# Autodesk Inventor assembly: diagonalstretcher_MIR
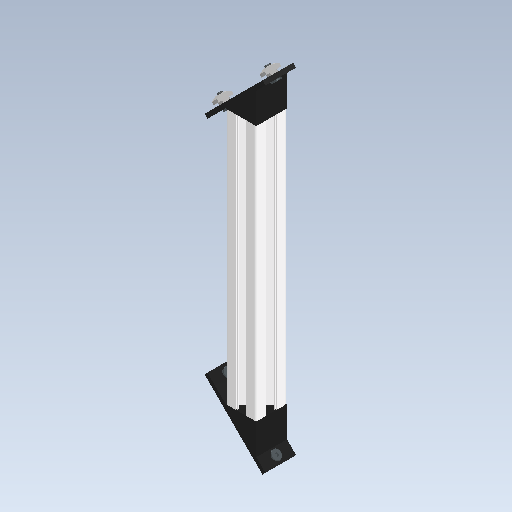
[picture p0: Inventor's stored thumbnail of the model, 512x512]
Saved by Autodesk Inventor 2020.2 (Build 242310000, 310)
## iProperties
Created: 2020-07-25
Part Number: diagonalstretcher_MIR
Document SubType Name: Assembly
Designer: JK
Author: JK
## Documents named in this file (3)
- C:\Users\JK\Documents\Inventor\Mesa\diagonalstretcher_MIR.iam
- C:\Users\JK\Documents\Inventor\Mesa\30x30x250_MIR.ipt
- C:\Users\JK\Documents\Inventor\Mesa\45degreebracketassembly_MIR.iam
## Components (3 placed, 2 different names)
1. 30x30x250_MIR:1 — Flush:1, Mate:3, Mate:1, Flush:2, Mate:4, Mate:2
2. 45degreebracketassembly_MIR:1 [sub-assembly] — Flush:1, Mate:3, Mate:1
3. 45degreebracketassembly_MIR:2 [sub-assembly] — Flush:2, Mate:4, Mate:2
## Relationships (6: Mate 4, Flush 2)
- Flush:1: 30x30x250_MIR:1 ↔ 45degreebracketassembly_MIR:1
- Mate:3: 30x30x250_MIR:1 ↔ 45degreebracketassembly_MIR:1
- Mate:1: 30x30x250_MIR:1 ↔ 45degreebracketassembly_MIR:1
- Flush:2: 30x30x250_MIR:1 ↔ 45degreebracketassembly_MIR:2
- Mate:4: 30x30x250_MIR:1 ↔ 45degreebracketassembly_MIR:2
- Mate:2: 30x30x250_MIR:1 ↔ 45degreebracketassembly_MIR:2
